# Autodesk Inventor assembly: 42146-04
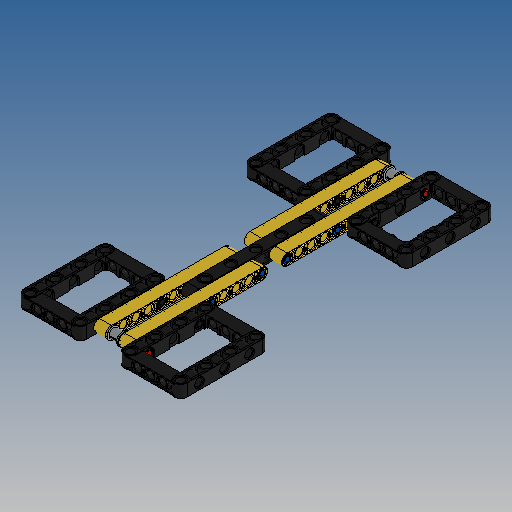
[picture p0: Inventor's stored thumbnail of the model, 512x512]
Saved by Autodesk Inventor 2025 (Build 290162010, 162A)
## iProperties
Created: 2024-11-14
Part Number: 42146-04
Material: Generisch
Document SubType Name: Assembly
Designer: hp.muther
Author: hp.muther
## Documents named in this file (8)
- D:\Inventor\Projekte\Muther\LEGO Technic\LEGO Technik - Raupenkran LR 13000 (42146)\42146-01-04.iam
- D:\Inventor\Projekte\Muther\LEGO Technic\LEGO Pieces\Pin's\6558-Blue.ipt
- D:\Inventor\Projekte\Muther\LEGO Technic\LEGO Pieces\Pin's\11214-Red.ipt
- D:\Inventor\Projekte\Muther\LEGO Technic\LEGO Pieces\Pin's\32054-LtBluishGray.ipt
- D:\Inventor\Projekte\Muther\LEGO Technic\LEGO Pieces\Pin's\2780-Black.ipt
- D:\Inventor\Projekte\Muther\LEGO Technic\LEGO Pieces\Lochbalken\32525-Yellow.ipt
- D:\Inventor\Projekte\Muther\LEGO Technic\LEGO Pieces\Rahmen, T-Stücke\64179-Black.ipt
- D:\Inventor\Projekte\Muther\LEGO Technic\LEGO Pieces\Lochbalken\73507-Black.ipt
## Components (21 placed, 7 different names)
1. 73507-Black:1 — Einfügen:1, Einfügen:2, Einfügen:3, Einfügen:4, Einfügen:11, Einfügen:12
2. 6558-Blue:1 — Einfügen:2, Passend:2
3. 6558-Blue:2 — Einfügen:3, Einfügen:5
4. 6558-Blue:3 — Einfügen:1, Passend:1
5. 6558-Blue:4 — Einfügen:4, Einfügen:6
6. 11214-Red:1 — Einfügen:7, Einfügen:8, Passend:8
7. 32054-LtBluishGray:1 — Einfügen:7, Passend:3, Passend:7
8. 2780-Black:1 — Einfügen:13
9. 2780-Black:2 — Einfügen:14
10. 2780-Black:3 — Einfügen:16
11. 2780-Black:4 — Einfügen:15
12. 32525-Yellow:1 — Einfügen:12, Passend:3, Einfügen:14, Einfügen:19
13. 32525-Yellow:2 — Einfügen:11, Passend:4, Einfügen:13, Einfügen:20
14. 32525-Yellow:3 — Einfügen:5, Passend:2, Einfügen:8, Einfügen:15, Einfügen:17
15. 32525-Yellow:4 — Einfügen:6, Passend:1, Einfügen:10, Einfügen:16, Einfügen:18
16. 64179-Black:1 — Einfügen:18, Passend:6
17. 64179-Black:2 — Einfügen:17, Passend:8
18. 64179-Black:3 — Einfügen:19, Passend:7
19. 64179-Black:4 — Einfügen:20, Passend:5
20. 11214-Red:2 — Einfügen:10, Passend:6
21. 32054-LtBluishGray:2 — Passend:4, Passend:5
## Relationships (28: Insert 20, Mate 8)
- Einfügen:1 [Insert]: 73507-Black:1 ↔ 6558-Blue:3
- Einfügen:2 [Insert]: 73507-Black:1 ↔ 6558-Blue:1
- Einfügen:3 [Insert]: 73507-Black:1 ↔ 6558-Blue:2
- Einfügen:4 [Insert]: 73507-Black:1 ↔ 6558-Blue:4
- Einfügen:5 [Insert]: 6558-Blue:2 ↔ 32525-Yellow:3
- Einfügen:6 [Insert]: 6558-Blue:4 ↔ 32525-Yellow:4
- Passend:1 [Mate]: 6558-Blue:3 ↔ 32525-Yellow:4
- Passend:2 [Mate]: 6558-Blue:1 ↔ 32525-Yellow:3
- Einfügen:7 [Insert]: 11214-Red:1 ↔ 32054-LtBluishGray:1
- Einfügen:8 [Insert]: 11214-Red:1 ↔ 32525-Yellow:3
- [Insert]: 11214-Red:2 ↔ 32054-LtBluishGray:2
- Einfügen:10 [Insert]: 32525-Yellow:4 ↔ 11214-Red:2
- Einfügen:11 [Insert]: 73507-Black:1 ↔ 32525-Yellow:2
- Einfügen:12 [Insert]: 73507-Black:1 ↔ 32525-Yellow:1
- Passend:3 [Mate]: 32054-LtBluishGray:1 ↔ 32525-Yellow:1
- Passend:4 [Mate]: 32525-Yellow:2 ↔ 32054-LtBluishGray:2
- Einfügen:13 [Insert]: 2780-Black:1 ↔ 32525-Yellow:2
- Einfügen:14 [Insert]: 2780-Black:2 ↔ 32525-Yellow:1
- Einfügen:15 [Insert]: 2780-Black:4 ↔ 32525-Yellow:3
- Einfügen:16 [Insert]: 2780-Black:3 ↔ 32525-Yellow:4
- Einfügen:17 [Insert]: 32525-Yellow:3 ↔ 64179-Black:2
- Einfügen:18 [Insert]: 32525-Yellow:4 ↔ 64179-Black:1
- Einfügen:19 [Insert]: 32525-Yellow:1 ↔ 64179-Black:3
- Einfügen:20 [Insert]: 32525-Yellow:2 ↔ 64179-Black:4
- Passend:5 [Mate]: 64179-Black:4 ↔ 32054-LtBluishGray:2
- Passend:6 [Mate]: 64179-Black:1 ↔ 11214-Red:2
- Passend:7 [Mate]: 32054-LtBluishGray:1 ↔ 64179-Black:3
- Passend:8 [Mate]: 11214-Red:1 ↔ 64179-Black:2
## Named parameters: d10_d8 = 0 mm
